# Autodesk Inventor assembly: Robot
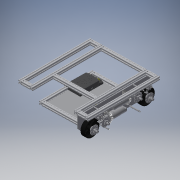
[picture p0: Inventor's stored thumbnail of the model, 180x180]
Saved by Autodesk Inventor 2017 (Build 210142000, 142)
## iProperties
Created: 2018-04-28
Part Number: Robot
Document SubType Name: Assembly
Designer: User
Author: User
## Documents named in this file (5)
- C:\Robotics\CAD\2018-19_CAD\Offseason\Robot.iam
- C:\Robotics\CAD\2018-19_CAD\Offseason\Frame.iam
- C:\Robotics\CAD\2018-19_CAD\InvertedDriveTrain.iam
- C:\Robotics\CAD\COTSParts\Rev\REV-31-1153RevHub.ipt
- C:\Robotics\CAD\2018-19_CAD\Offseason\Electronics Plate.ipt
## Components (5 placed, 4 different names)
1. Frame:1 [sub-assembly] — Mate:1, Flush:1, Flush:2, Mate:2, Mate:3, Flush:3
2. InvertedDriveTrain:2 [sub-assembly] — Mate:1, Flush:1, Flush:2
3. REV-31-1153RevHub:2 — Mate:4
4. Electronics Plate:1 — Mate:2, Mate:3, Flush:3, Mate:4, Mate:5
5. REV-31-1153RevHub:3 — Mate:5
## Relationships (8: Mate 5, Flush 3)
- Mate:1: Frame:1 ↔ InvertedDriveTrain:2
- Flush:1: Frame:1 ↔ InvertedDriveTrain:2
- Flush:2: Frame:1 ↔ InvertedDriveTrain:2
- Mate:2: Frame:1 ↔ Electronics Plate:1
- Mate:3: Frame:1 ↔ Electronics Plate:1
- Flush:3: Frame:1 ↔ Electronics Plate:1
- Mate:4: REV-31-1153RevHub:2 ↔ Electronics Plate:1
- Mate:5: Electronics Plate:1 ↔ REV-31-1153RevHub:3
